# Autodesk Inventor assembly: tower and bucket
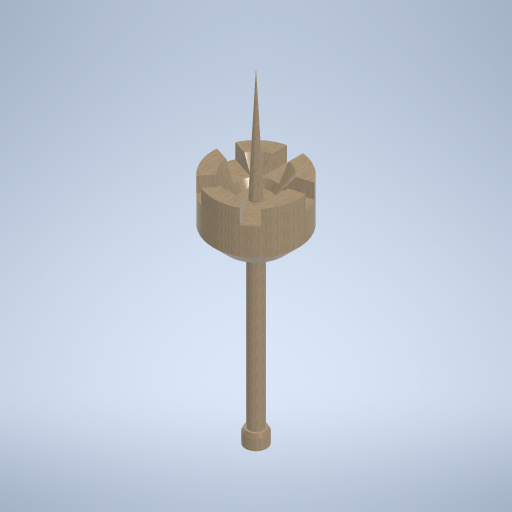
[picture p0: Inventor's stored thumbnail of the model, 512x512]
Saved by Autodesk Inventor 2023 (Build 270158000, 158)
## iProperties
Created: 2023-10-27
Part Number: tower and bucket
Document SubType Name: Assembly
Designer: Admin
Author: Admin
## Documents named in this file (4)
- C:\Users\Admin\Desktop\tower and bucket.iam
- C:\Users\Admin\Desktop\Tower.ipt
- C:\Users\Admin\Desktop\bucket.ipt
- C:\Users\Admin\Desktop\trianglef.ipt
## Components (3 placed, 3 different names)
1. Tower:1 — Rotational:1, Rotational:2
2. trianglef:1 — Rotational:2
3. bucket:1 — Rotational:1
## Relationships (2: RevoluteJoint 2)
- Rotational:1 [RevoluteJoint]: Tower:1 ↔ bucket:1
- Rotational:2 [RevoluteJoint]: Tower:1 ↔ trianglef:1
